# Autodesk Inventor assembly: PiShelf
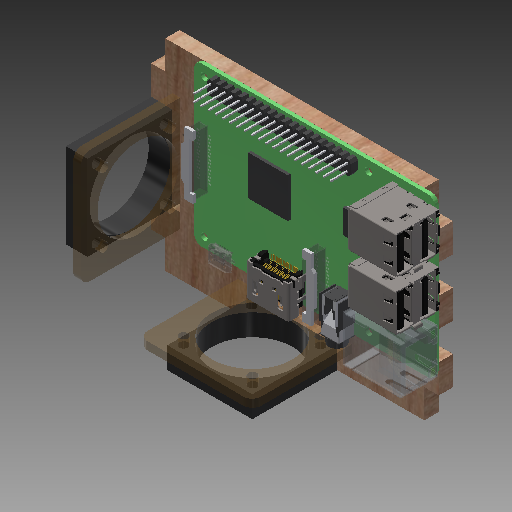
[picture p0: Inventor's stored thumbnail of the model, 512x512]
Saved by Autodesk Inventor 2019 (Build 230136000, 136)
## iProperties
Created: 2019-01-17
Part Number: PiShelf
Document SubType Name: Assembly
Designer: nxgam
Author: nxgam
## Documents named in this file (5)
- C:\Users\nxgam\Documents\CAD\Inventor\DiscoDraw\PiShelf.iam
- C:\Users\nxgam\Documents\CAD\Inventor\DiscoDraw\PiShelf.ipt
- C:\Users\nxgam\Documents\CAD\Inventor\DiscoDraw\Imported\Pi Fan.ipt
- C:\Users\nxgam\Documents\CAD\Inventor\DiscoDraw\FanMount.ipt
- C:\Users\nxgam\Documents\CAD\Inventor\DiscoDraw\Imported\raspberry-pi-2-model-b-3d-cad-assembly-model-2.snapshot.20\RaspberryPi2 STEP214.ipt
## Components (6 placed, 4 different names)
1. PiShelf:1 — Flush:1, Flush:2, Mate:1, Mate:2, Flush:7, Mate:5, Mate:6, Mate:7, Mate:8, Mate:9, Flush:8, Flush:9
2. Pi Fan:1 — Flush:2, Mate:1, Mate:3, Mate:5
3. Pi Fan:2 — Flush:1, Mate:2, Mate:4, Mate:7
4. FanMount:1 — Flush:6, Mate:4, Flush:7, Mate:8
5. FanMount:2 — Mate:3, Flush:6, Mate:6
6. RaspberryPi2 STEP214:1 — Mate:9, Flush:8, Flush:9
## Relationships (15: Mate 9, Flush 6)
- Flush:1: PiShelf:1 ↔ Pi Fan:2
- Flush:2: PiShelf:1 ↔ Pi Fan:1
- Mate:1: PiShelf:1 ↔ Pi Fan:1
- Mate:2: PiShelf:1 ↔ Pi Fan:2
- Mate:3: Pi Fan:1 ↔ FanMount:2
- Flush:6: FanMount:1 ↔ FanMount:2
- Mate:4: Pi Fan:2 ↔ FanMount:1
- Flush:7: PiShelf:1 ↔ FanMount:1
- Mate:5: PiShelf:1 ↔ Pi Fan:1
- Mate:6: PiShelf:1 ↔ FanMount:2
- Mate:7: PiShelf:1 ↔ Pi Fan:2
- Mate:8: PiShelf:1 ↔ FanMount:1
- Mate:9: PiShelf:1 ↔ RaspberryPi2 STEP214:1
- Flush:8: PiShelf:1 ↔ RaspberryPi2 STEP214:1
- Flush:9: PiShelf:1 ↔ RaspberryPi2 STEP214:1
